# Autodesk Inventor assembly: DriveAssembly
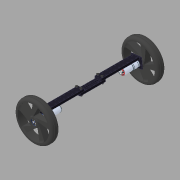
[picture p0: Inventor's stored thumbnail of the model, 180x180]
Saved by Autodesk Inventor 2017 (Build 210142000, 142)
## iProperties
Created: 2017-05-07
Part Number: DriveAssembly
Document SubType Name: Assembly
Designer: zallen
Author: zallen
## Documents named in this file (15)
- C:\Users\zallen\Documents\Autodesk Inventor Projects\LaundryRobot_v0.1\Base\Drive Wheel Assembly\DriveAssembly.iam
- C:\Users\zallen\Documents\Autodesk Inventor Projects\Makeblock\Beam0824-144-Blue.ipt
- C:\Users\zallen\Documents\Autodesk Inventor Projects\Makeblock\Beam0824-096-Blue.ipt
- C:\Users\zallen\Documents\Autodesk Inventor Projects\LaundryRobot_v0.1\Base\Drive Wheel Assembly\DriveAssembly\Design Accelerator\Bolted Connection1.iam
- C:\Users\zallen\Documents\Autodesk Inventor Projects\LaundryRobot_v0.1\Base\Drive Wheel Assembly\DriveAssembly\Design Accelerator\Bolted Connection2.iam
- C:\Users\zallen\Documents\Autodesk Inventor Projects\LaundryRobot_v0.1\Base\Drive Wheel Assembly\DriveAssembly\Design Accelerator\Bolted Connection3.iam
- C:\Users\zallen\Documents\Autodesk Inventor Projects\LaundryRobot_v0.1\Base\Drive Wheel Assembly\DriveAssembly\Design Accelerator\Bolted Connection4.iam
- C:\Users\zallen\Documents\Autodesk Inventor Projects\Makeblock\DC Motor-25 Bracket B-Blue.ipt
- C:\Users\zallen\Documents\Autodesk Inventor Projects\LaundryRobot_v0.1\Base\Drive Wheel Assembly\DriveAssembly\Design Accelerator\Bolted Connection5.iam
- C:\Users\zallen\Documents\Autodesk Inventor Projects\LaundryRobot_v0.1\Base\Drive Wheel Assembly\DriveAssembly\Design Accelerator\Bolted Connection6.iam
- C:\Users\zallen\Documents\Autodesk Inventor Projects\LaundryRobot_v0.1\Base\Drive Wheel Assembly\DriveAssembly\Design Accelerator\Bolted Connection7.iam
- C:\Users\zallen\Documents\Autodesk Inventor Projects\LaundryRobot_v0.1\Base\Drive Wheel Assembly\DriveAssembly\Design Accelerator\Bolted Connection8.iam
- C:\Users\zallen\Documents\Autodesk Inventor Projects\DC Motor with Encoder\Motor.ipt
- C:\Users\zallen\Documents\Autodesk Inventor Projects\Pololu\Wheel-144×29.ipt
- C:\Users\zallen\Documents\Autodesk Inventor Projects\Pololu\WheelAdapter-4mm\WheelAdapter-4mm.iam
## Components (19 placed, 7 different names)
1. Beam0824-144-Blue:1 — Mate:1, Mate:2, Mate:3, Mate:7, Mate:8, Mate:9, Mate:10, Mate:15, Mate:16, Mate:17
2. Beam0824-144-Blue:2 — Mate:4, Mate:5, Mate:6, Mate:11, Mate:12, Mate:13, Mate:14, Mate:22, Mate:23, Mate:24
3. Beam0824-096-Blue:1 — Mate:1, Mate:2, Mate:3, Mate:4, Mate:5, Mate:6
4. Bolted Connection:1 [sub-assembly] — Mate:7, Mate:8
5. Bolted Connection:2 [sub-assembly] — Mate:9, Mate:10
6. Bolted Connection:3 [sub-assembly] — Mate:11, Mate:12
7. Bolted Connection:4 [sub-assembly] — Mate:13, Mate:14
8. DC Motor-25 Bracket B-Blue:1 — Mate:15, Mate:16, Mate:17, Mate:18, Mate:19, Mate:20, Mate:21, Mate:32, Mate:33
9. DC Motor-25 Bracket B-Blue:2 — Mate:22, Mate:23, Mate:24, Mate:25, Mate:26, Mate:27, Mate:28, Mate:30, Mate:31, Mate:39
10. Bolted Connection:5 [sub-assembly] — Mate:18, Mate:19
11. Bolted Connection:6 [sub-assembly] — Mate:20, Mate:21
12. Bolted Connection:7 [sub-assembly] — Mate:25, Mate:26
13. Bolted Connection:8 [sub-assembly] — Mate:27, Mate:28
14. Motor:1 — Mate:30, Mate:31, Mate:34
15. Motor:2 — Mate:32, Mate:33, Mate:35, Mate:42
16. Wheel-144×29:1 — Mate:34, Mate:37, Mate:38
17. Wheel-144×29:2 — Mate:35, Mate:41, Mate:40
18. WheelAdapter-4mm:1 [sub-assembly] — Mate:37, Mate:38, Mate:39
19. WheelAdapter-4mm:2 [sub-assembly] — Mate:41, Mate:40, Mate:42
## Relationships (40: Mate 40)
- Mate:1: Beam0824-144-Blue:1 ↔ Beam0824-096-Blue:1
- Mate:2: Beam0824-144-Blue:1 ↔ Beam0824-096-Blue:1
- Mate:3: Beam0824-144-Blue:1 ↔ Beam0824-096-Blue:1
- Mate:4: Beam0824-144-Blue:2 ↔ Beam0824-096-Blue:1
- Mate:5: Beam0824-144-Blue:2 ↔ Beam0824-096-Blue:1
- Mate:6: Beam0824-144-Blue:2 ↔ Beam0824-096-Blue:1
- Mate:7: Beam0824-144-Blue:1 ↔ Bolted Connection:1
- Mate:8: Beam0824-144-Blue:1 ↔ Bolted Connection:1
- Mate:9: Beam0824-144-Blue:1 ↔ Bolted Connection:2
- Mate:10: Beam0824-144-Blue:1 ↔ Bolted Connection:2
- Mate:11: Beam0824-144-Blue:2 ↔ Bolted Connection:3
- Mate:12: Beam0824-144-Blue:2 ↔ Bolted Connection:3
- Mate:13: Beam0824-144-Blue:2 ↔ Bolted Connection:4
- Mate:14: Beam0824-144-Blue:2 ↔ Bolted Connection:4
- Mate:15: Beam0824-144-Blue:1 ↔ DC Motor-25 Bracket B-Blue:1
- Mate:16: Beam0824-144-Blue:1 ↔ DC Motor-25 Bracket B-Blue:1
- Mate:17: Beam0824-144-Blue:1 ↔ DC Motor-25 Bracket B-Blue:1
- Mate:18: DC Motor-25 Bracket B-Blue:1 ↔ Bolted Connection:5
- Mate:19: DC Motor-25 Bracket B-Blue:1 ↔ Bolted Connection:5
- Mate:20: DC Motor-25 Bracket B-Blue:1 ↔ Bolted Connection:6
- Mate:21: DC Motor-25 Bracket B-Blue:1 ↔ Bolted Connection:6
- Mate:22: Beam0824-144-Blue:2 ↔ DC Motor-25 Bracket B-Blue:2
- Mate:23: Beam0824-144-Blue:2 ↔ DC Motor-25 Bracket B-Blue:2
- Mate:24: Beam0824-144-Blue:2 ↔ DC Motor-25 Bracket B-Blue:2
- Mate:25: DC Motor-25 Bracket B-Blue:2 ↔ Bolted Connection:7
- Mate:26: DC Motor-25 Bracket B-Blue:2 ↔ Bolted Connection:7
- Mate:27: DC Motor-25 Bracket B-Blue:2 ↔ Bolted Connection:8
- Mate:28: DC Motor-25 Bracket B-Blue:2 ↔ Bolted Connection:8
- Mate:30: DC Motor-25 Bracket B-Blue:2 ↔ Motor:1
- Mate:31: DC Motor-25 Bracket B-Blue:2 ↔ Motor:1
- Mate:32: DC Motor-25 Bracket B-Blue:1 ↔ Motor:2
- Mate:33: DC Motor-25 Bracket B-Blue:1 ↔ Motor:2
- Mate:34: Motor:1 ↔ Wheel-144×29:1
- Mate:35: Motor:2 ↔ Wheel-144×29:2
- Mate:37: Wheel-144×29:1 ↔ WheelAdapter-4mm:1
- Mate:38: Wheel-144×29:1 ↔ WheelAdapter-4mm:1
- Mate:39: DC Motor-25 Bracket B-Blue:2 ↔ WheelAdapter-4mm:1
- Mate:41: Wheel-144×29:2 ↔ WheelAdapter-4mm:2
- Mate:40: Wheel-144×29:2 ↔ WheelAdapter-4mm:2
- Mate:42: Motor:2 ↔ WheelAdapter-4mm:2
